# Autodesk Inventor assembly: ГЛАЗ НОВЫЙ СБОРКА_ЗЕРКАЛО
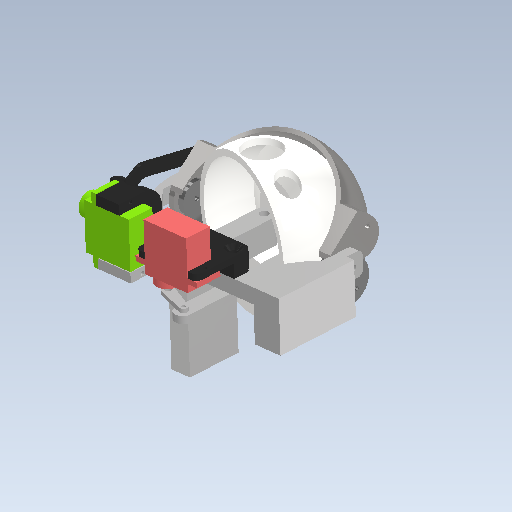
[picture p0: Inventor's stored thumbnail of the model, 512x512]
Saved by Autodesk Inventor 2020 (Build 240168000, 168)
## iProperties
Created: 2022-02-16
Part Number: ГЛАЗ НОВЫЙ СБОРКА_ЗЕРКАЛО
Document SubType Name: Assembly
Designer: Администратор
Author: Администратор
## Documents named in this file (14)
- \\sch239.net\UserHomes\Students\Other\glazovaes\3D\Onstage\Face\ГЛАЗ НОВЫЙ СБОРКА_ЗЕРКАЛО.iam
- \\sch239.net\UserHomes\Students\Other\glazovaes\3D\Onstage\Face\шатун движенияглаза_ЗЕРКАЛО.ipt
- \\sch239.net\UserHomes\Students\Other\glazovaes\3D\Onstage\Face\связующий сервы движения глаз_ЗЕРКАЛО.ipt
- \\sch239.net\UserHomes\Students\Other\glazovaes\3D\Onstage\Face\связующий сервы век_ЗЕРКАЛО.ipt
- \\sch239.net\UserHomes\Students\Other\glazovaes\3D\Onstage\Face\нижнее веко_ЗЕРКАЛО.ipt
- \\sch239.net\UserHomes\Students\Other\glazovaes\3D\Onstage\Face\держалка сервы движения глаз_ЗЕРКАЛО.ipt
- \\sch239.net\UserHomes\Students\Other\glazovaes\3D\Onstage\Face\держалка сервы век_ЗЕРКАЛО.ipt
- \\sch239.net\UserHomes\Students\Other\glazovaes\3D\Onstage\Face\держалка глаза_ЗЕРКАЛО.ipt
- \\sch239.net\UserHomes\Students\Other\glazovaes\3D\Onstage\Face\верхнее веко_ЗЕРКАЛО.ipt
- \\sch239.net\UserHomes\Students\Other\glazovaes\3D\Onstage\Face\SERVO_ЗЕРКАЛО.ipt
- \\sch239.net\UserHomes\Students\Other\glazovaes\3D\Onstage\Face\нижний шатун век_ЗЕРКАЛО.ipt
- \\sch239.net\UserHomes\Students\Other\glazovaes\3D\Onstage\Face\зрачок_ЗЕРКАЛО.ipt
- \\sch239.net\UserHomes\Students\Other\glazovaes\3D\Onstage\Face\белок глаза_ЗЕРКАЛО_ЗЕРКАЛО.ipt
- \\sch239.net\UserHomes\Students\Other\glazovaes\3D\Onstage\Face\верхний шатун века_ЗЕРКАЛО1_ЗЕРКАЛО.ipt
## Components (14 placed, 13 different names)
1. шатун движенияглаза_ЗЕРКАЛО:1 — Совмещение:31, Совмещение:30, Совмещение:47, Совмещение:46
2. связующий сервы движения глаз_ЗЕРКАЛО:1 — Совмещение:43, Совмещение:20, Совмещение:16, Совмещение:44
3. связующий сервы век_ЗЕРКАЛО:1 — Совмещение:31, Совмещение:30, Совмещение:38
4. нижнее веко_ЗЕРКАЛО:1 — Совмещение:7, Совмещение:6, Совмещение:5, Совмещение:9, Совмещение:8, Совмещение:42, Совмещение:41
5. держалка сервы движения глаз_ЗЕРКАЛО:1 — Совмещение:34, Совмещение:33, Совмещение:32, Совмещение:37, Совмещение:36, Совмещение:35
6. держалка сервы век_ЗЕРКАЛО:1 — Совмещение:23, Совмещение:22, Совмещение:21
7. держалка глаза_ЗЕРКАЛО:1 — Совмещение:34, Совмещение:33, Совмещение:32, Совмещение:7, Совмещение:6, Совмещение:5, Совмещение:10, Совмещение:19, Совмещение:18, Угол:1, Совмещение:48, Совмещение:45
8. верхнее веко_ЗЕРКАЛО:1 — Совмещение:10, Совмещение:9, Совмещение:8, Совмещение:14, Совмещение:13
9. SERVO_ЗЕРКАЛО:1 — Совмещение:43, Совмещение:23, Совмещение:22, Совмещение:21, Совмещение:20, Совмещение:19, Совмещение:18, Угол:1
10. SERVO_ЗЕРКАЛО:2 — Совмещение:38, Совмещение:37, Совмещение:36, Совмещение:35
11. нижний шатун век_ЗЕРКАЛО:1 — Совмещение:16, Совмещение:14, Совмещение:13
12. зрачок_ЗЕРКАЛО:1 — Совмещение:40, Совмещение:39
13. белок глаза_ЗЕРКАЛО_ЗЕРКАЛО:1 — Совмещение:48, Совмещение:47, Совмещение:46, Совмещение:45, Совмещение:40, Совмещение:39
14. верхний шатун века_ЗЕРКАЛО1_ЗЕРКАЛО:1 — Совмещение:44, Совмещение:42, Совмещение:41
## Relationships (35: Mate 34, Angle 1)
- Совмещение:31 [Mate]: шатун движенияглаза_ЗЕРКАЛО:1 ↔ связующий сервы век_ЗЕРКАЛО:1
- Совмещение:30 [Mate]: шатун движенияглаза_ЗЕРКАЛО:1 ↔ связующий сервы век_ЗЕРКАЛО:1
- Совмещение:34 [Mate]: держалка сервы движения глаз_ЗЕРКАЛО:1 ↔ держалка глаза_ЗЕРКАЛО:1
- Совмещение:33 [Mate]: держалка сервы движения глаз_ЗЕРКАЛО:1 ↔ держалка глаза_ЗЕРКАЛО:1
- Совмещение:32 [Mate]: держалка сервы движения глаз_ЗЕРКАЛО:1 ↔ держалка глаза_ЗЕРКАЛО:1
- Совмещение:7 [Mate]: нижнее веко_ЗЕРКАЛО:1 ↔ держалка глаза_ЗЕРКАЛО:1
- Совмещение:6 [Mate]: нижнее веко_ЗЕРКАЛО:1 ↔ держалка глаза_ЗЕРКАЛО:1
- Совмещение:5 [Mate]: нижнее веко_ЗЕРКАЛО:1 ↔ держалка глаза_ЗЕРКАЛО:1
- Совмещение:10 [Mate]: держалка глаза_ЗЕРКАЛО:1 ↔ верхнее веко_ЗЕРКАЛО:1
- Совмещение:9 [Mate]: нижнее веко_ЗЕРКАЛО:1 ↔ верхнее веко_ЗЕРКАЛО:1
- Совмещение:8 [Mate]: нижнее веко_ЗЕРКАЛО:1 ↔ верхнее веко_ЗЕРКАЛО:1
- Совмещение:43 [Mate]: связующий сервы движения глаз_ЗЕРКАЛО:1 ↔ SERVO_ЗЕРКАЛО:1
- Совмещение:23 [Mate]: держалка сервы век_ЗЕРКАЛО:1 ↔ SERVO_ЗЕРКАЛО:1
- Совмещение:22 [Mate]: держалка сервы век_ЗЕРКАЛО:1 ↔ SERVO_ЗЕРКАЛО:1
- Совмещение:21 [Mate]: держалка сервы век_ЗЕРКАЛО:1 ↔ SERVO_ЗЕРКАЛО:1
- Совмещение:20 [Mate]: связующий сервы движения глаз_ЗЕРКАЛО:1 ↔ SERVO_ЗЕРКАЛО:1
- Совмещение:19 [Mate]: держалка глаза_ЗЕРКАЛО:1 ↔ SERVO_ЗЕРКАЛО:1
- Совмещение:18 [Mate]: держалка глаза_ЗЕРКАЛО:1 ↔ SERVO_ЗЕРКАЛО:1
- Совмещение:38 [Mate]: связующий сервы век_ЗЕРКАЛО:1 ↔ SERVO_ЗЕРКАЛО:2
- Совмещение:37 [Mate]: держалка сервы движения глаз_ЗЕРКАЛО:1 ↔ SERVO_ЗЕРКАЛО:2
- Совмещение:36 [Mate]: держалка сервы движения глаз_ЗЕРКАЛО:1 ↔ SERVO_ЗЕРКАЛО:2
- Совмещение:35 [Mate]: держалка сервы движения глаз_ЗЕРКАЛО:1 ↔ SERVO_ЗЕРКАЛО:2
- Совмещение:16 [Mate]: связующий сервы движения глаз_ЗЕРКАЛО:1 ↔ нижний шатун век_ЗЕРКАЛО:1
- Совмещение:14 [Mate]: верхнее веко_ЗЕРКАЛО:1 ↔ нижний шатун век_ЗЕРКАЛО:1
- Совмещение:13 [Mate]: верхнее веко_ЗЕРКАЛО:1 ↔ нижний шатун век_ЗЕРКАЛО:1
- Угол:1 [Angle] (0 deg): держалка глаза_ЗЕРКАЛО:1 ↔ SERVO_ЗЕРКАЛО:1
- Совмещение:48 [Mate]: держалка глаза_ЗЕРКАЛО:1 ↔ белок глаза_ЗЕРКАЛО_ЗЕРКАЛО:1
- Совмещение:47 [Mate]: шатун движенияглаза_ЗЕРКАЛО:1 ↔ белок глаза_ЗЕРКАЛО_ЗЕРКАЛО:1
- Совмещение:46 [Mate]: шатун движенияглаза_ЗЕРКАЛО:1 ↔ белок глаза_ЗЕРКАЛО_ЗЕРКАЛО:1
- Совмещение:45 [Mate]: держалка глаза_ЗЕРКАЛО:1 ↔ белок глаза_ЗЕРКАЛО_ЗЕРКАЛО:1
- Совмещение:40 [Mate]: зрачок_ЗЕРКАЛО:1 ↔ белок глаза_ЗЕРКАЛО_ЗЕРКАЛО:1
- Совмещение:39 [Mate]: зрачок_ЗЕРКАЛО:1 ↔ белок глаза_ЗЕРКАЛО_ЗЕРКАЛО:1
- Совмещение:44 [Mate]: связующий сервы движения глаз_ЗЕРКАЛО:1 ↔ верхний шатун века_ЗЕРКАЛО1_ЗЕРКАЛО:1
- Совмещение:42 [Mate]: нижнее веко_ЗЕРКАЛО:1 ↔ верхний шатун века_ЗЕРКАЛО1_ЗЕРКАЛО:1
- Совмещение:41 [Mate]: нижнее веко_ЗЕРКАЛО:1 ↔ верхний шатун века_ЗЕРКАЛО1_ЗЕРКАЛО:1
